# Autodesk Inventor assembly: TailAssembly
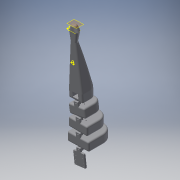
[picture p0: Inventor's stored thumbnail of the model, 180x180]
Saved by Autodesk Inventor 2018 (Build 220112000, 112)
## iProperties
Created: 2018-10-19
Part Number: TailAssembly
Document SubType Name: Assembly
Designer: reide
Author: reide
## Documents named in this file (8)
- C:\Users\reide\OneDrive\Documents\Inventor\TSA\2019\Animatronics\Glyptodon\Glyptodon Work\TailAssembly.iam
- C:\Users\reide\OneDrive\Documents\Inventor\TSA\2019\Animatronics\Glyptodon\Glyptodon Work\Tail\Tail4.ipt
- C:\Users\reide\OneDrive\Documents\Inventor\TSA\2019\Animatronics\Glyptodon\Glyptodon Work\Tail\Tail_Mount.ipt
- C:\Users\reide\OneDrive\Documents\Inventor\TSA\2019\Animatronics\Glyptodon\Glyptodon Work\Tail\Tail3.ipt
- C:\Users\reide\OneDrive\Documents\Inventor\TSA\2019\Animatronics\Glyptodon\Glyptodon Work\Tail\Tail5.ipt
- C:\Users\reide\OneDrive\Documents\Inventor\TSA\2019\Animatronics\Glyptodon\Glyptodon Work\Tail\Tail6.ipt
- C:\Users\reide\OneDrive\Documents\Inventor\TSA\2019\Animatronics\Glyptodon\Glyptodon Work\Tail\Club1.ipt
- C:\Users\reide\OneDrive\Documents\Inventor\TSA\2019\Animatronics\Glyptodon\Glyptodon Work\Tail\Club2.ipt
## Components (7 placed, 7 different names)
1. Tail_Mount:1 — Mate:7, Mate:8
2. Tail3:1 — Mate:1, Mate:4, Mate:7, Mate:8
3. Tail4:2 — Mate:1, Mate:2, Mate:4, Mate:5
4. Tail5:1 — Mate:2, Mate:3, Mate:5, Mate:6
5. Tail6:1 — Mate:3, Mate:6, Flush:1, Flush:2
6. Club1:1 — Flush:1, Flush:2, Flush:3, Flush:4
7. Club2:1 — Flush:3, Flush:4
## Relationships (12: Mate 8, Flush 4)
- Mate:1: Tail3:1 ↔ Tail4:2
- Mate:2: Tail4:2 ↔ Tail5:1
- Mate:3: Tail5:1 ↔ Tail6:1
- Mate:4: Tail3:1 ↔ Tail4:2
- Mate:5: Tail4:2 ↔ Tail5:1
- Mate:6: Tail5:1 ↔ Tail6:1
- Mate:7: Tail_Mount:1 ↔ Tail3:1
- Mate:8: Tail_Mount:1 ↔ Tail3:1
- Flush:1: Tail6:1 ↔ Club1:1
- Flush:2 (25 mm): Tail6:1 ↔ Club1:1
- Flush:3: Club1:1 ↔ Club2:1
- Flush:4 (15 mm): Club1:1 ↔ Club2:1
